# Autodesk Inventor assembly: frame-and-walls
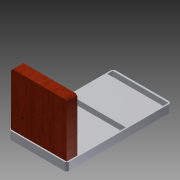
[picture p0: Inventor's stored thumbnail of the model, 180x180]
Saved by Autodesk Inventor 2015 (Build 190159000, 159)
## iProperties
Created: 2014-07-16
Part Number: frame-and-walls
Document SubType Name: Assembly
Designer: pc
Author: pc
## Documents named in this file (3)
- C:\Users\pc\Documents\blinds\openscad\frame-and-walls.iam
- C:\Users\pc\Documents\blinds\openscad\base-frame.ipt
- C:\Users\pc\Documents\blinds\openscad\wall-front.ipt
## Components (2 placed, 2 different names)
1. base-frame:1 — Mate:1, Mate:2, Mate:3
2. Front wall:1 — Mate:1, Mate:2, Mate:3
## Relationships (3: Mate 3)
- Mate:1: base-frame:1 ↔ Front wall:1
- Mate:2: base-frame:1 ↔ Front wall:1
- Mate:3: base-frame:1 ↔ Front wall:1
